# Autodesk Inventor assembly: Battery Pack
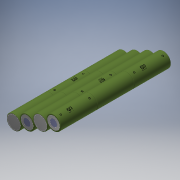
[picture p0: Inventor's stored thumbnail of the model, 180x180]
Saved by Autodesk Inventor 2019.2 (Build 232265000, 265)
## iProperties
Created: 2018-12-05
Part Number: Battery Pack
Document SubType Name: Assembly
Designer: Petar
Author: Petar
## Documents named in this file (2)
- D:\OMG\E-Board\CAD\Inventor\Electrical Components\Battery Pack - A123.iam
- D:\OMG\E-Board\CAD\Inventor\Electrical Components\Battery Cell - A123.ipt
## Components (12 placed, 1 different names)
1. Battery Cell - A123:1 — Rigid:1, Rigid:2, Tangent:1
2. Battery Cell - A123:2 — Rigid:1, Flush:1, Mate:4
3. Battery Cell - A123:3 — Rigid:2
4. Battery Cell - A123:4 — Tangent:1, Tangent:2
5. Battery Cell - A123:5
6. Battery Cell - A123:6 — Flush:1, Flush:2, Planar:1, Mate:10
7. Battery Cell - A123:7 — Tangent:2, Tangent:3
8. Battery Cell - A123:8 — Flush:2, Flush:3, Planar:1, Mate:11
9. Battery Cell - A123:9
10. Battery Cell - A123:10 — Tangent:3
11. Battery Cell - A123:11
12. Battery Cell - A123:12 — Flush:3, Mate:7
## Relationships (24: WeldJoint 8, Mate 8, Flush 4, Tangent 3, PlanarJoint 1)
- Rigid:1 [WeldJoint]: Battery Cell - A123:1 ↔ Battery Cell - A123:2
- Rigid:2 [WeldJoint]: Battery Cell - A123:1 ↔ Battery Cell - A123:3
- [WeldJoint]: Battery Cell - A123:4 ↔ Battery Cell - A123:5
- [WeldJoint]: Battery Cell - A123:4 ↔ Battery Cell - A123:6
- [WeldJoint]: Battery Cell - A123:7 ↔ Battery Cell - A123:8
- [WeldJoint]: Battery Cell - A123:7 ↔ Battery Cell - A123:9
- [WeldJoint]: Battery Cell - A123:10 ↔ Battery Cell - A123:11
- [WeldJoint]: Battery Cell - A123:10 ↔ Battery Cell - A123:12
- Tangent:1: Battery Cell - A123:1 ↔ Battery Cell - A123:4
- Flush:1: Battery Cell - A123:2 ↔ Battery Cell - A123:6
- Tangent:2: Battery Cell - A123:4 ↔ Battery Cell - A123:7
- Flush:2: Battery Cell - A123:6 ↔ Battery Cell - A123:8
- Tangent:3: Battery Cell - A123:7 ↔ Battery Cell - A123:10
- Flush:3: Battery Cell - A123:8 ↔ Battery Cell - A123:12
- Mate:4: Battery Cell - A123:2
- Mate:7: Battery Cell - A123:12
- Mate:8
- Mate:9
- Planar:1: Battery Cell - A123:6 ↔ Battery Cell - A123:8
- Mate:10: Battery Cell - A123:6
- Mate:11: Battery Cell - A123:8
- Mate:12
- Mate:13
- Flush:4
## Named parameters: d2_d0 = 0 mm, d3_d1 = 0 mm, d4_d0 = 0 mm, d5_d1 = 0 mm, d6_d0 = 0 mm, d7_d1 = 0 mm
